# Autodesk Inventor assembly: gapura_case
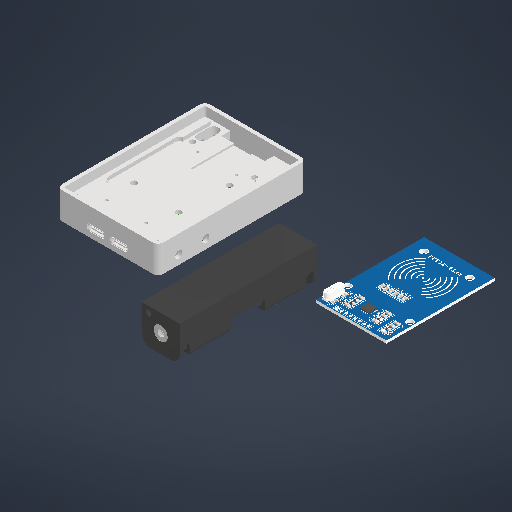
[picture p0: Inventor's stored thumbnail of the model, 512x512]
Saved by Autodesk Inventor 2026.4 (Build 304435000, 435)
## iProperties
Created: 2026-10-02
Part Number: gapura_case
Document SubType Name: Assembly
Designer: LENOVO
Author: LENOVO
## Documents named in this file (5)
- C:\Users\LENOVO\OneDrive - ACTVET (Abu Dhabi Center for Technical and Vocational Education and Training)\99-Projects\claude\Wireless RFID Reader\3d\gapura_case.iam
- C:\Users\LENOVO\OneDrive - ACTVET (Abu Dhabi Center for Technical and Vocational Education and Training)\99-Projects\claude\Wireless RFID Reader\3d\ESP32-C5-WIFI6-KIT-N16R8-3d_20260304\ESP32-C5-WIFI6-KIT-N16R8-.iam
- C:\Users\LENOVO\OneDrive - ACTVET (Abu Dhabi Center for Technical and Vocational Education and Training)\99-Projects\claude\Wireless RFID Reader\3d\18650 1x Holder - Compressed\18650 1x Holder - Compressed.ipt
- C:\Users\LENOVO\OneDrive - ACTVET (Abu Dhabi Center for Technical and Vocational Education and Training)\99-Projects\claude\Wireless RFID Reader\3d\RFID_Reader\RFID_Reader.ipt
- C:\Users\LENOVO\OneDrive - ACTVET (Abu Dhabi Center for Technical and Vocational Education and Training)\99-Projects\claude\Wireless RFID Reader\3d\gapura_case_pt1.ipt
## Components (4 placed, 4 different names)
1. 18650 1x Holder - Compressed:1
2. RFID_Reader:1
3. gapura_case_pt1:1 — Mate:1, Flush:1, Mate:2
4. ESP32-C5-WIFI6-KIT-N16R8-:2 [sub-assembly] — Mate:1, Flush:1, Mate:2
## Relationships (3: Mate 2, Flush 1)
- Mate:1 (0.25 mm): gapura_case_pt1:1 ↔ ESP32-C5-WIFI6-KIT-N16R8-:2
- Flush:1: gapura_case_pt1:1 ↔ ESP32-C5-WIFI6-KIT-N16R8-:2
- Mate:2 (0.28 mm): gapura_case_pt1:1 ↔ ESP32-C5-WIFI6-KIT-N16R8-:2
